# Autodesk Inventor assembly: RJ45 Jack
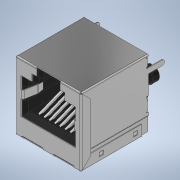
[picture p0: Inventor's stored thumbnail of the model, 180x180]
Saved by Autodesk Inventor 2020.1 (Build 241239000, 239)
## iProperties
Created: 2019-12-05
Part Number: RJ45 Jack
Document SubType Name: Assembly
Designer: S. Lee
Mass: 5.69665 g
Surface Area: 64.3586 cm^2
Volume: 2.72387 cm^3
Density: 2.09138 g/cm^3
Author: S. Lee
## Documents named in this file (6)
- X:\AutoDesk\InventorProjects\Library\Electrical\Connectors\Comercial Connectors\RJ45\RJ45 Jack.iam
- X:\AutoDesk\InventorProjects\Library\Electrical\Connectors\Comercial Connectors\RJ45\Parts\RJ45 Lower Insert.ipt
- X:\AutoDesk\InventorProjects\Library\Electrical\Connectors\Comercial Connectors\RJ45\Parts\RJ45 Odd Pins.ipt
- X:\AutoDesk\InventorProjects\Library\Electrical\Connectors\Comercial Connectors\RJ45\Parts\RJ45 Main Insert.ipt
- X:\AutoDesk\InventorProjects\Library\Electrical\Connectors\Comercial Connectors\RJ45\Parts\RJ45 Shell.ipt
- X:\AutoDesk\InventorProjects\Library\Electrical\Connectors\Comercial Connectors\RJ45\Parts\RJ45 Even Pins.ipt
## Components (11 placed, 5 different names)
1. RJ45 Lower Insert:1 — Mate:1, Mate:2, Mate:3, Slider:1, Mate:4, Mate:6, Mate:8, Mate:9, Mate:10, Mate:11, Mate:12, Mate:13, Mate:14, Mate:15, Mate:16, Mate:17, Mate:18, Mate:19, Mate:23, Mate:24, Mate:25, Mate:26, Mate:27, Mate:28, Mate:29, Mate:30, Mate:31
2. RJ45 Odd Pins:1 — Mate:1, Mate:2, Mate:3
3. RJ45 Odd Pins:2 — Mate:10, Mate:13, Mate:18
4. RJ45 Odd Pins:3 — Mate:12, Mate:15, Mate:16
5. RJ45 Odd Pins:4 — Mate:11, Mate:14, Mate:17
6. RJ45 Even Pins:1 — Mate:8, Mate:9, Mate:19
7. RJ45 Even Pins:2 — Mate:23, Mate:24, Mate:27
8. RJ45 Even Pins:3 — Mate:29, Mate:30, Mate:31
9. RJ45 Even Pins:4 — Mate:25, Mate:26, Mate:28
10. RJ45 Main Insert:1 — Slider:1, Mate:4, Mate:5, Mate:7
11. RJ45 Shell:1 — Mate:5, Mate:6, Mate:7
## Relationships (29: Mate 28, TranslationJoint 1)
- Mate:1: RJ45 Lower Insert:1 ↔ RJ45 Odd Pins:1
- Mate:2: RJ45 Lower Insert:1 ↔ RJ45 Odd Pins:1
- Mate:3: RJ45 Lower Insert:1 ↔ RJ45 Odd Pins:1
- Slider:1 [TranslationJoint]: RJ45 Lower Insert:1 ↔ RJ45 Main Insert:1
- Mate:4: RJ45 Lower Insert:1 ↔ RJ45 Main Insert:1
- Mate:5: RJ45 Main Insert:1 ↔ RJ45 Shell:1
- Mate:6: RJ45 Lower Insert:1 ↔ RJ45 Shell:1
- Mate:7: RJ45 Main Insert:1 ↔ RJ45 Shell:1
- Mate:8: RJ45 Lower Insert:1 ↔ RJ45 Even Pins:1
- Mate:9: RJ45 Lower Insert:1 ↔ RJ45 Even Pins:1
- Mate:10: RJ45 Lower Insert:1 ↔ RJ45 Odd Pins:2
- Mate:11: RJ45 Lower Insert:1 ↔ RJ45 Odd Pins:4
- Mate:12: RJ45 Lower Insert:1 ↔ RJ45 Odd Pins:3
- Mate:13: RJ45 Lower Insert:1 ↔ RJ45 Odd Pins:2
- Mate:14: RJ45 Lower Insert:1 ↔ RJ45 Odd Pins:4
- Mate:15: RJ45 Lower Insert:1 ↔ RJ45 Odd Pins:3
- Mate:16: RJ45 Lower Insert:1 ↔ RJ45 Odd Pins:3
- Mate:17: RJ45 Lower Insert:1 ↔ RJ45 Odd Pins:4
- Mate:18: RJ45 Lower Insert:1 ↔ RJ45 Odd Pins:2
- Mate:19: RJ45 Lower Insert:1 ↔ RJ45 Even Pins:1
- Mate:23: RJ45 Lower Insert:1 ↔ RJ45 Even Pins:2
- Mate:24: RJ45 Lower Insert:1 ↔ RJ45 Even Pins:2
- Mate:25: RJ45 Lower Insert:1 ↔ RJ45 Even Pins:4
- Mate:26: RJ45 Lower Insert:1 ↔ RJ45 Even Pins:4
- Mate:27: RJ45 Lower Insert:1 ↔ RJ45 Even Pins:2
- Mate:28: RJ45 Lower Insert:1 ↔ RJ45 Even Pins:4
- Mate:29: RJ45 Lower Insert:1 ↔ RJ45 Even Pins:3
- Mate:30: RJ45 Lower Insert:1 ↔ RJ45 Even Pins:3
- Mate:31: RJ45 Lower Insert:1 ↔ RJ45 Even Pins:3
